# Autodesk Inventor assembly: Pata - Ensamble_MIR
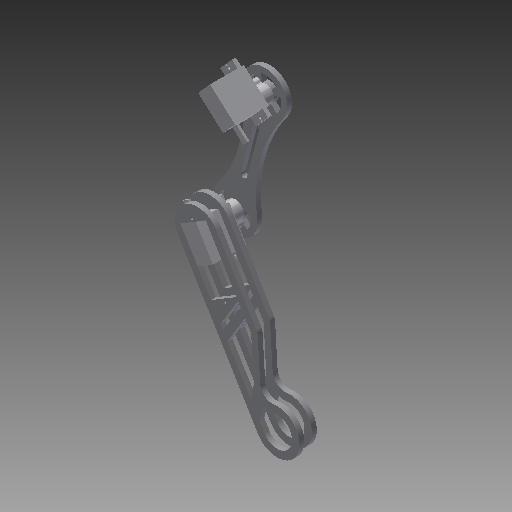
[picture p0: Inventor's stored thumbnail of the model, 512x512]
Saved by Autodesk Inventor 2019 (Build 230136000, 136)
## iProperties
Created: 2020-02-12
Part Number: Pata - Ensamble_MIR
Document SubType Name: Assembly
Designer: eddysanoli
Mass: 47.369 g
Surface Area: 327.582 cm^2
Volume: 47.369 cm^3
Density: 1 g/cm^3
Author: jacqu
## Documents named in this file (4)
- C:\Users\jacqu\Desktop\Robotica1_Proyecto-Cuadrupedo-master\Robotica1-Proyecto_Cuadrupedo\Pata - Ensamble_MIR.iam
- C:\Users\jacqu\Desktop\Robotica1_Proyecto-Cuadrupedo-master\Robotica1-Proyecto_Cuadrupedo\Pata - Antebrazo_MIR.ipt
- C:\Users\jacqu\Desktop\Robotica1_Proyecto-Cuadrupedo-master\Robotica1-Proyecto_Cuadrupedo\Pata - Brazo_MIR.ipt
- C:\Users\jacqu\Desktop\Robotica1_Proyecto-Cuadrupedo-master\Robotica1-Proyecto_Cuadrupedo\Servo - Componente_MIR.ipt
## Components (5 placed, 3 different names)
1. Pata - Antebrazo_MIR:1 — Coincidencia:17, Coincidencia:13, Coincidencia:16, Coincidencia:15
2. Pata - Brazo_MIR:1 — Coincidencia:8, Coincidencia:7, Coincidencia:1
3. Servo - Componente_MIR:1 — Coincidencia:17, Coincidencia:13, Coincidencia:8, Coincidencia:7, Coincidencia:1, Nivelación:1, Coincidencia:10, Coincidencia:9
4. Servo - Componente_MIR:2 — Coincidencia:16, Coincidencia:15
5. Pata - Brazo_MIR:2 — Nivelación:1, Coincidencia:10, Coincidencia:9
## Relationships (10: Mate 9, Flush 1)
- Coincidencia:17 [Mate]: Pata - Antebrazo_MIR:1 ↔ Servo - Componente_MIR:1
- Coincidencia:13 [Mate]: Pata - Antebrazo_MIR:1 ↔ Servo - Componente_MIR:1
- Coincidencia:8 [Mate]: Pata - Brazo_MIR:1 ↔ Servo - Componente_MIR:1
- Coincidencia:7 [Mate]: Pata - Brazo_MIR:1 ↔ Servo - Componente_MIR:1
- Coincidencia:1 [Mate]: Pata - Brazo_MIR:1 ↔ Servo - Componente_MIR:1
- Coincidencia:16 [Mate]: Pata - Antebrazo_MIR:1 ↔ Servo - Componente_MIR:2
- Coincidencia:15 [Mate]: Pata - Antebrazo_MIR:1 ↔ Servo - Componente_MIR:2
- Nivelación:1 [Flush]: Servo - Componente_MIR:1 ↔ Pata - Brazo_MIR:2
- Coincidencia:10 [Mate]: Servo - Componente_MIR:1 ↔ Pata - Brazo_MIR:2
- Coincidencia:9 [Mate]: Servo - Componente_MIR:1 ↔ Pata - Brazo_MIR:2
